# Autodesk Inventor assembly: DiaD Front Bumper
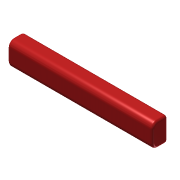
[picture p0: Inventor's stored thumbnail of the model, 180x180]
Saved by Autodesk Inventor 2013 (Build 170138000, 138)
## iProperties
Created: 2013-05-20
Part Number: DiaD Front Bumper
Document SubType Name: Assembly
Designer: Nemo
Author: Nemo
## Documents named in this file (6)
- H:\Nemo\Documents\Robotics\COTS Parts\Drive in a Day\DiaD Front Bumper.iam
- H:\Nemo\Documents\Robotics\COTS Parts\Drive in a Day\217-2593-016 Rev2 Bumper Mount Front.ipt
- H:\Nemo\Documents\Robotics\COTS Parts\Drive in a Day\FrontBumpers.ipt
- H:\Nemo\Documents\Robotics\COTS Parts\Drive in a Day\DiaD bumper fastener subassy.iam
- H:\Nemo\Documents\Robotics\COTS Parts\Fasteners\14-20 BHCS x750.ipt
- H:\Nemo\Documents\Robotics\COTS Parts\Fasteners\14-20 locknut.ipt
## Components (15 placed, 5 different names)
1. 217-2593-016 Rev2 Bumper Mount Front:1 — Insert:5, Insert:6, Insert:8, Insert:10, Insert:11, Insert:14
2. 217-2593-016 Rev2 Bumper Mount Front:2 — Mate:2, Mate:3, Insert:7, Insert:9, Insert:12, Insert:13
3. FrontBumpers:1
4. DiaD bumper fastener subassy:1 [sub-assembly]
5. DiaD bumper fastener subassy:2 [sub-assembly] — Mate:2, Mate:3
6. DiaD bumper fastener subassy:3 [sub-assembly] — Insert:6
7. DiaD bumper fastener subassy:4 [sub-assembly] — Insert:5
8. 14-20 BHCS x750:1 — Insert:7
9. 14-20 BHCS x750:2 — Insert:8
10. 14-20 BHCS x750:3 — Insert:12
11. 14-20 BHCS x750:4 — Insert:11
12. 14-20 locknut:1 — Insert:9
13. 14-20 locknut:2 — Insert:10
14. 14-20 locknut:3 — Insert:14
15. 14-20 locknut:4 — Insert:13
## Relationships (14: Insert 11, Mate 3)
- [Mate]: 217-2593-016 Rev2 Bumper Mount Front:1 ↔ FrontBumpers:1
- [Insert]: 217-2593-016 Rev2 Bumper Mount Front:2 ↔ DiaD bumper fastener subassy:1
- Mate:2: 217-2593-016 Rev2 Bumper Mount Front:2 ↔ DiaD bumper fastener subassy:2
- Mate:3: 217-2593-016 Rev2 Bumper Mount Front:2 ↔ DiaD bumper fastener subassy:2
- Insert:5: 217-2593-016 Rev2 Bumper Mount Front:1 ↔ DiaD bumper fastener subassy:4
- Insert:6: 217-2593-016 Rev2 Bumper Mount Front:1 ↔ DiaD bumper fastener subassy:3
- Insert:7: 217-2593-016 Rev2 Bumper Mount Front:2 ↔ 14-20 BHCS x750:1
- Insert:8: 217-2593-016 Rev2 Bumper Mount Front:1 ↔ 14-20 BHCS x750:2
- Insert:9 (4.445 mm): 217-2593-016 Rev2 Bumper Mount Front:2 ↔ 14-20 locknut:1
- Insert:10 (4.445 mm): 217-2593-016 Rev2 Bumper Mount Front:1 ↔ 14-20 locknut:2
- Insert:11: 217-2593-016 Rev2 Bumper Mount Front:1 ↔ 14-20 BHCS x750:4
- Insert:12: 217-2593-016 Rev2 Bumper Mount Front:2 ↔ 14-20 BHCS x750:3
- Insert:13 (3.175 mm): 217-2593-016 Rev2 Bumper Mount Front:2 ↔ 14-20 locknut:4
- Insert:14 (3.175 mm): 217-2593-016 Rev2 Bumper Mount Front:1 ↔ 14-20 locknut:3
